# Autodesk Inventor assembly: Single Acting Piston With Hardware
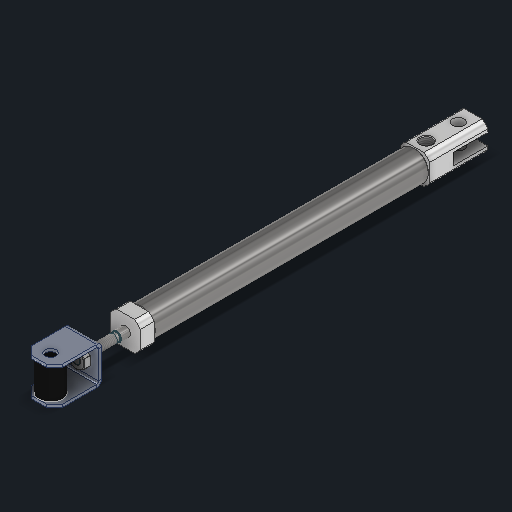
[picture p0: Inventor's stored thumbnail of the model, 512x512]
Saved by Autodesk Inventor 2025.1 (Build 291241000, 241)
## iProperties
Created: 2022-09-23
Part Number: Single Acting Piston With Hardware
Document SubType Name: Assembly
Designer: maxxw
Mass: 12.2112 g
Surface Area: 100.21 cm^2
Volume: 12.2112 cm^3
Density: 1 g/cm^3
Author: maxxw
## Documents named in this file (7)
- C:\Users\avere\VEX\High Stakes\CAD\ROBOPROS-CAD-Inventor\Motion\Pneumatics\Single Acting Piston With Hardware.iam
- C:\Users\avere\VEX\High Stakes\CAD\ROBOPROS-CAD-Inventor\Motion\Pneumatics\Reference Parts\Pistons\Single Acting Piston Rod.ipt
- C:\Users\avere\VEX\High Stakes\CAD\ROBOPROS-CAD-Inventor\Motion\Pneumatics\Reference Parts\Pistons\Single Acting Piston Body.ipt
- C:\Users\avere\VEX\High Stakes\CAD\ROBOPROS-CAD-Inventor\Motion\Pneumatics\Cylinder Mount.ipt
- C:\Users\avere\VEX\High Stakes\CAD\ROBOPROS-CAD-Inventor\Structure\Hardware\Nut Hex #6-32.ipt
- C:\Users\avere\VEX\High Stakes\CAD\ROBOPROS-CAD-Inventor\Motion\Spacers\Spacer Nylon .375 OD\NSpacer .375 OD x .500.ipt
- C:\Users\avere\VEX\High Stakes\CAD\ROBOPROS-CAD-Inventor\Motion\Spacers\Spacer Nylon .375 OD.ipt
## Components (6 placed, 5 different names)
1. Single Acting Piston Rod:1 — Mate:1, Mate:2, Insert:4
2. Single Acting Piston Body:1 — Mate:1, Mate:2
3. Cylinder Mount:1
4. Nut Hex #6-32:1
5. Nut Hex #6-32:2 — Insert:4
6. NSpacer .375 OD x .500:1
## Relationships (6: Insert 4, Mate 2)
- Mate:1: Single Acting Piston Rod:1 ↔ Single Acting Piston Body:1
- Mate:2: Single Acting Piston Rod:1 ↔ Single Acting Piston Body:1
- [Insert]: Cylinder Mount:1 ↔ Nut Hex #6-32:2
- [Insert]: Cylinder Mount:1 ↔ Nut Hex #6-32:1
- [Insert]: Cylinder Mount:1 ↔ NSpacer .375 OD x .500:1
- Insert:4: Single Acting Piston Rod:1 ↔ Nut Hex #6-32:2
## Named parameters: d13_d0 = 0 mm
